# Autodesk Inventor assembly: RailWheelSys
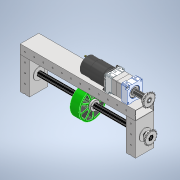
[picture p0: Inventor's stored thumbnail of the model, 180x180]
Saved by Autodesk Inventor 2022 (Build 260153000, 153)
## iProperties
Created: 2022-01-14
Part Number: RailWheelSys
Document SubType Name: Assembly
Designer: tagaz
Author: tagaz
## Documents named in this file (9)
- C:\Users\Ty Gazaway\Documents\t3-cad\CAD\2022 Parts\RailWheelSys.iam
- C:\Users\Ty Gazaway\Documents\t3-cad\CAD\2022 Parts\Generic\RailSupp.ipt
- C:\Users\Ty Gazaway\Documents\t3-cad\CAD\Bearing  for THUNDER.ipt
- C:\Users\Ty Gazaway\Documents\t3-cad\CAD\2022 Parts\Generic\railThunder.ipt
- C:\Users\Ty Gazaway\Documents\t3-cad\CAD\2022 Parts\Generic\3in Compliance wheel.ipt
- C:\Users\Ty Gazaway\Documents\t3-cad\CAD\2022 Parts\16T Alum Hub Sprock 25 Chain.ipt
- C:\Users\Ty Gazaway\Documents\t3-cad\CAD\Hex Shaft Collar.ipt
- C:\Users\Ty Gazaway\Documents\t3-cad\CAD\2022 Parts\Generic\RailSupp2.ipt
- C:\Users\Ty Gazaway\Documents\t3-cad\CAD\Generic and Stock\VersaPlanetary Parts\VersaPlanetary Two Stage 775.iam
## Components (14 placed, 8 different names)
1. RailSupp:1 — Mate:1, Flush:1, Flush:2, Insert:1, Insert:2, Mate:6, Flush:5, Mate:15, Flush:6
2. RailSupp:2 — Mate:1, Flush:1, Flush:2, Insert:3, Insert:4
3. Bearing  for THUNDER:1 — Insert:1
4. Bearing  for THUNDER:2 — Insert:2, Flush:3, Mate:2, Mate:3
5. Bearing  for THUNDER:3 — Insert:3
6. Bearing  for THUNDER:4 — Insert:4
7. railThunder:1 — Flush:3, Mate:2, Mate:3, Mate:4, Mate:5, Flush:4, Mate:7, Mate:8, Mate:9, Mate:10, Mate:13, Mate:14, Flush:8
8. 3in Compliance wheel:1 — Mate:4, Mate:5, Mate:6, Mate:11, Mate:12
9. 16T Alum Hub Sprock 25 Chain:1 — Flush:4, Mate:7, Mate:8
10. Hex Shaft Collar:1 — Mate:9, Mate:10, Mate:11
11. Hex Shaft Collar:2 — Mate:12, Mate:13, Mate:14
12. RailSupp2:1 — Flush:5, Mate:15, Flush:6, Mate:16, Flush:7
13. VersaPlanetary Two Stage 775:1 [sub-assembly] — Mate:16, Flush:7, Flush:8, Flush:9, Mate:17, Mate:18
14. 16T Alum Hub Sprock 25 Chain:2 — Flush:9, Mate:17, Mate:18
## Relationships (31: Mate 18, Flush 9, Insert 4)
- Mate:1 (266.7 mm): RailSupp:1 ↔ RailSupp:2
- Flush:1: RailSupp:1 ↔ RailSupp:2
- Flush:2: RailSupp:1 ↔ RailSupp:2
- Insert:1: RailSupp:1 ↔ Bearing  for THUNDER:1
- Insert:2: RailSupp:1 ↔ Bearing  for THUNDER:2
- Insert:3: RailSupp:2 ↔ Bearing  for THUNDER:3
- Insert:4: RailSupp:2 ↔ Bearing  for THUNDER:4
- Flush:3: Bearing  for THUNDER:2 ↔ railThunder:1
- Mate:2: Bearing  for THUNDER:2 ↔ railThunder:1
- Mate:3: Bearing  for THUNDER:2 ↔ railThunder:1
- Mate:4: railThunder:1 ↔ 3in Compliance wheel:1
- Mate:5: railThunder:1 ↔ 3in Compliance wheel:1
- Mate:6 (123.825 mm): RailSupp:1 ↔ 3in Compliance wheel:1
- Flush:4: railThunder:1 ↔ 16T Alum Hub Sprock 25 Chain:1
- Mate:7: railThunder:1 ↔ 16T Alum Hub Sprock 25 Chain:1
- Mate:8: railThunder:1 ↔ 16T Alum Hub Sprock 25 Chain:1
- Mate:9: railThunder:1 ↔ Hex Shaft Collar:1
- Mate:10: railThunder:1 ↔ Hex Shaft Collar:1
- Mate:11: 3in Compliance wheel:1 ↔ Hex Shaft Collar:1
- Mate:12: 3in Compliance wheel:1 ↔ Hex Shaft Collar:2
- Mate:13: railThunder:1 ↔ Hex Shaft Collar:2
- Mate:14: railThunder:1 ↔ Hex Shaft Collar:2
- Flush:5: RailSupp:1 ↔ RailSupp2:1
- Mate:15: RailSupp:1 ↔ RailSupp2:1
- Flush:6: RailSupp:1 ↔ RailSupp2:1
- Mate:16: RailSupp2:1 ↔ VersaPlanetary Two Stage 775:1
- Flush:7: RailSupp2:1 ↔ VersaPlanetary Two Stage 775:1
- Flush:8: railThunder:1 ↔ VersaPlanetary Two Stage 775:1
- Flush:9: VersaPlanetary Two Stage 775:1 ↔ 16T Alum Hub Sprock 25 Chain:2
- Mate:17: VersaPlanetary Two Stage 775:1 ↔ 16T Alum Hub Sprock 25 Chain:2
- Mate:18: VersaPlanetary Two Stage 775:1 ↔ 16T Alum Hub Sprock 25 Chain:2
